# Autodesk Inventor assembly: ALPHA_001160_Electrode 8
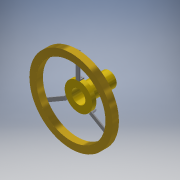
[picture p0: Inventor's stored thumbnail of the model, 180x180]
Saved by Autodesk Inventor 2017 (Build 210142000, 142)
## iProperties
Created: 2015-11-18
Part Number: ALPHA_001160_Electrode 8
Document SubType Name: Assembly
Designer: massen
Author: massen
## Documents named in this file (4)
- E:\Vault\Designs\Positrons\Accumulator\Accumulator Penning Trap\ALPHA_001160_Electrode 8.iam
- E:\Vault\Designs\Positrons\Accumulator\Accumulator Penning Trap\ALPHA_001158_Electrode8-mountring.ipt
- E:\Vault\Designs\Positrons\Accumulator\Accumulator Penning Trap\ALPHA_001158_Electrode8-mountbracket.ipt
- E:\Vault\Designs\Positrons\Accumulator\Accumulator Penning Trap\ALPHA_001157_EndNosePiece.ipt
## Components (5 placed, 3 different names)
1. ALPHA_001158_Electrode8-mountring:1 — Mate:1, Mate:2, Mate:3, Mate:5, Mate:7, Mate:8
2. ALPHA_001158_Electrode8-mountbracket:1 — Mate:1, Mate:2, Mate:4
3. ALPHA_001157_EndNosePiece:1 — Mate:3, Mate:4, Mate:6, Mate:9
4. ALPHA_001158_Electrode8-mountbracket:2 — Mate:5, Mate:6
5. ALPHA_001158_Electrode8-mountbracket:3 — Mate:7, Mate:8, Mate:9
## Relationships (9: Mate 9)
- Mate:1: ALPHA_001158_Electrode8-mountring:1 ↔ ALPHA_001158_Electrode8-mountbracket:1
- Mate:2: ALPHA_001158_Electrode8-mountring:1 ↔ ALPHA_001158_Electrode8-mountbracket:1
- Mate:3: ALPHA_001158_Electrode8-mountring:1 ↔ ALPHA_001157_EndNosePiece:1
- Mate:4: ALPHA_001158_Electrode8-mountbracket:1 ↔ ALPHA_001157_EndNosePiece:1
- Mate:5: ALPHA_001158_Electrode8-mountring:1 ↔ ALPHA_001158_Electrode8-mountbracket:2
- Mate:6: ALPHA_001157_EndNosePiece:1 ↔ ALPHA_001158_Electrode8-mountbracket:2
- Mate:7: ALPHA_001158_Electrode8-mountring:1 ↔ ALPHA_001158_Electrode8-mountbracket:3
- Mate:8: ALPHA_001158_Electrode8-mountring:1 ↔ ALPHA_001158_Electrode8-mountbracket:3
- Mate:9: ALPHA_001157_EndNosePiece:1 ↔ ALPHA_001158_Electrode8-mountbracket:3
